# Autodesk Inventor assembly: Front Right Foot
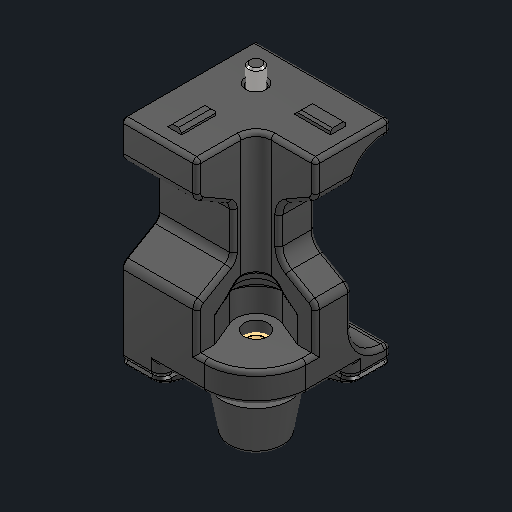
[picture p0: Inventor's stored thumbnail of the model, 512x512]
Saved by Autodesk Inventor 2025.1 (Build 291241020, 241B)
## iProperties
Created: 2025-05-09
Part Number: Front Right Foot
Document SubType Name: Assembly
Designer: AdminForWorker
Title: Front Right Foot
Author: AdminForWorker
## Documents named in this file (9)
- C:\Users\Joshua Eah\Documents\Voron 0.2\CAD\Master Assembly\Skirt\Feet\Front Right Foot.iam
- C:\Users\Joshua Eah\Documents\Voron 0.2\CAD\Master Assembly\Skirt\Feet\Rubber Foot.ipt
- C:\Users\Joshua Eah\Documents\Voron 0.2\CAD\Master Assembly\Hardware\M3x40 BHCS.ipt
- C:\Users\Joshua Eah\Documents\Voron 0.2\CAD\Master Assembly\Hardware\M2x10 Self Tapper.ipt
- C:\Users\Joshua Eah\Documents\Voron 0.2\CAD\Master Assembly\Hardware\M3x10 BHCS.ipt
- C:\Users\Joshua Eah\Documents\Voron 0.2\CAD\Master Assembly\Hardware\M3 Threaded Insert.ipt
- C:\Users\Joshua Eah\Documents\Voron 0.2\CAD\Master Assembly\Skirt\Feet\Front Right Foot (1).ipt
- C:\Users\Joshua Eah\Documents\Voron 0.2\CAD\Master Assembly\Skirt\Feet\Foot Accent Mirrored.ipt
- Foot Accent Left.ipt
## Components (8 placed, 7 different names)
1. Front Right Foot:1
2. Foot Accent:1
3. Rubber Foot:3
4. M3x40 BHCS:1
5. M2x10 Self Tapper:1
6. M2x10 Self Tapper:2
7. M3x10 BHCS:1
8. M3 Threaded Insert:1
## Relationships (2: Insert 2)
- [Insert]: Foot Accent:1 ↔ M2x10 Self Tapper:1
- [Insert]: Foot Accent:1 ↔ M2x10 Self Tapper:2
